# Autodesk Inventor assembly: Base-Rotation-Test
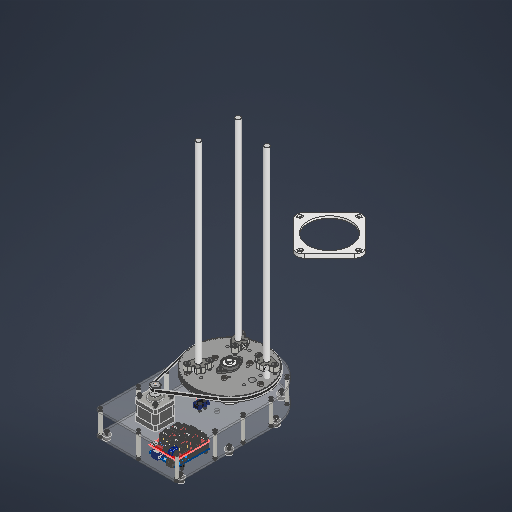
[picture p0: Inventor's stored thumbnail of the model, 512x512]
Saved by Autodesk Inventor 2025.2 (Build 292293000, 293)
## iProperties
Created: 2025-04-10
Part Number: Base-Rotation-Test
Document SubType Name: Assembly
Designer: Tiago
Author: Tiago
## Documents named in this file (32)
- C:\Users\Tiago\Documents\Inventor\Exp. Braço v1\Base-Rotation-Test.iam
- C:\Users\Tiago\Documents\Inventor\Exp. Braço v1\NEMA17 42-38.ipt
- C:\Users\Tiago\Documents\Inventor\Exp. Braço v1\Linear_Shaft_Support_SHF10.ipt
- C:\Users\Tiago\Documents\Inventor\Exp. Braço v1\rodshaft_10x400.ipt
- C:\Users\Tiago\Documents\Inventor\Exp. Braço v1\Arduino_CNC_Assembly.iam
- C:\Users\Tiago\Documents\Inventor\Exp. Braço v1\Base_solida_Down.ipt
- C:\Users\Tiago\Documents\Inventor\Exp. Braço v1\Amortecedor_Borracha.ipt
- C:\Users\Tiago\Documents\Inventor\Exp. Braço v1\Espaçador_m3_L3.5.ipt
- C:\Users\Tiago\Documents\Inventor\Exp. Braço v1\espaçador_M3_L40.ipt
- C:\Users\Tiago\Documents\Inventor\Exp. Braço v1\GT2Pulley_z20.ipt
- C:\Users\Tiago\Documents\Inventor\Exp. Braço v1\Base-Rotation\Design Accelerator\Synchronous Belts Transmission3.iam
- C:\Users\Tiago\Documents\Inventor\Exp. Braço v1\Anilha_M3.ipt
- C:\Users\Tiago\Documents\Inventor\Exp. Braço v1\M3 x0.5 ALT (...).ipt
- C:\Users\Tiago\Documents\Inventor\Exp. Braço v1\Porca_sextavada(4M).ipt
- C:\Users\Tiago\Documents\Inventor\Exp. Braço v1\M3 x8L_hexagonal_BigHEAD.ipt
- C:\Users\Tiago\Documents\Inventor\Exp. Braço v1\M3 x5L_hexagonal.ipt
- C:\Users\Tiago\Documents\Inventor\Exp. Braço v1\M4x22L_Hex.ipt
- C:\Users\Tiago\Documents\Inventor\Exp. Braço v1\M5 x12L_Hex_C.ipt
- M5 x12L_Hex_C.ipt
- C:\Users\Tiago\Documents\Inventor\Exp. Braço v1\M5x16L_Hex.ipt
- C:\Users\Tiago\Documents\Inventor\Exp. Braço v1\Porca_sextavada(3M).ipt
- C:\Users\Tiago\Documents\Inventor\Exp. Braço v1\M2x12L_Hex.ipt
- M2x12L_Hex.ipt
- C:\Users\Tiago\Documents\Inventor\Exp. Braço v1\Porca_sextavada(M2).ipt
- C:\Users\Tiago\Documents\Inventor\Exp. Braço v1\M5_nylonLock_Nut.ipt
- C:\Users\Tiago\Documents\Inventor\Exp. Braço v1\Limit switch\complete limit switch\complete limit switch\complete limit switch.ipt
- C:\Users\Tiago\Documents\Inventor\Exp. Braço v1\Base_solida_TestBR.ipt
- C:\Users\Tiago\Documents\Inventor\Exp. Braço v1\Rolamento TestBR\61814\61814\61814.iam
- C:\Users\Tiago\Documents\Inventor\Exp. Braço v1\Test_BR\Fix_bearing_Base.ipt
- C:\Users\Tiago\Documents\Inventor\Exp. Braço v1\PoliaDentada220dentes_TestBR.ipt
- C:\Users\Tiago\Documents\Inventor\Exp. Braço v1\Test_BR\Fix_toDown_bearing.ipt
- C:\Users\Tiago\Documents\Inventor\Exp. Braço v1\KFL08 - Mancal Flange oval Ø8_BRTest.ipt
## Components (124 placed, 29 different names)
1. NEMA17 42-38:1 — Mate:85, Mate:86, Flush:4, Mate:87, Flush:8
2. Linear_Shaft_Support_SHF10:1 — Mate:20, Insert:129, Insert:138, Insert:139
3. Linear_Shaft_Support_SHF10:2 — Mate:21, Mate:133, Insert:131, Insert:134, Insert:135
4. Linear_Shaft_Support_SHF10:3 — Mate:22, Insert:130, Insert:136, Insert:137
5. rodshaft_10x400:1 — Mate:22
6. rodshaft_10x400:2 — Mate:21, Mate:133
7. rodshaft_10x400:3 — Mate:20
8. Base_solida_TestBR:1 — Mate:31, Flush:1, Flush:2, Mate:85, Mate:87, Mate:97, Mate:98, Flush:8, Mate:107, Mate:111, Mate:112, Mate:113, Mate:117, Insert:150, Insert:151, Insert:162, Insert:163, Insert:164, Insert:165, Insert:166, Insert:167, Insert:168, Insert:169, Insert:170, Insert:171, Insert:172, Insert:173, Mate:184, Mate:185, Mate:186, Mate:190, Flush:9, Mate:192, Mate:193
9. Arduino_CNC_Assembly:1 [sub-assembly] — Mate:32, Mate:33, Mate:34, Mate:35, Mate:36, Insert:111, Insert:114, Insert:115, Insert:116
10. Base_solida_Down:1 — Mate:31, Flush:1, Flush:2, Mate:32, Mate:33, Mate:34, Mate:35, Mate:36, Mate:37, Mate:38, Mate:39, Mate:40, Mate:41, Mate:42, Mate:43, Mate:44, Mate:54, Mate:55, Mate:56, Mate:57, Mate:58, Mate:59, Mate:61, Mate:62, Mate:63, Mate:64, Mate:65, Mate:66, Mate:67, Mate:68, Mate:69, Mate:70, Mate:71, Mate:72, Mate:73, Mate:74, Mate:75, Mate:76, Mate:77, Mate:78, Mate:79, Mate:80, Mate:81, Mate:82, Mate:83, Mate:84, Flush:7, Mate:153, Mate:154, Insert:95, Insert:96, Mate:155, Mate:156, Mate:157, Mate:158, Mate:159, Mate:160, Mate:161, Mate:162, Insert:112, Insert:113, Insert:140, Insert:141, Insert:142, Insert:143, Insert:144, Insert:145, Insert:146, Insert:147, Insert:152, Insert:153, Insert:154, Insert:155, Insert:156, Insert:157, Insert:158, Insert:159, Insert:160, Insert:161, Insert:175, Insert:176
11. Amortecedor_Borracha:1 — Mate:57, Mate:159, Insert:102
12. Amortecedor_Borracha:2 — Mate:58, Mate:160, Insert:100
13. Amortecedor_Borracha:3 — Mate:59, Mate:161, Insert:99
14. Amortecedor_Borracha:4 — Mate:56, Mate:158, Insert:101
15. Amortecedor_Borracha:5 — Mate:153, Mate:162, Insert:98
16. Amortecedor_Borracha:6 — Mate:54, Mate:156, Mate:164
17. Amortecedor_Borracha:7 — Mate:154, Mate:155, Insert:97
18. Amortecedor_Borracha:8 — Mate:55, Mate:157, Mate:163
19. Espaçador_m3_L3.5:1 — Mate:37, Mate:41
20. Espaçador_m3_L3.5:2 — Mate:38, Mate:44
21. Espaçador_m3_L3.5:3 — Mate:40, Mate:42
22. Espaçador_m3_L3.5:4 — Mate:39, Mate:43
23. espaçador_M3_L40:1 — Mate:61, Mate:73
24. espaçador_M3_L40:2 — Mate:62, Mate:75
25. espaçador_M3_L40:3 — Mate:63, Mate:76
26. espaçador_M3_L40:4 — Mate:64, Mate:77
27. espaçador_M3_L40:5 — Mate:65, Mate:78
28. espaçador_M3_L40:6 — Mate:66, Mate:79
29. espaçador_M3_L40:7 — Mate:67, Mate:74
30. espaçador_M3_L40:8 — Mate:68, Mate:84
31. espaçador_M3_L40:9 — Mate:69, Mate:83
32. espaçador_M3_L40:10 — Mate:70, Mate:82
33. espaçador_M3_L40:11 — Mate:71, Mate:81
34. espaçador_M3_L40:12 — Mate:72, Mate:80
35. GT2Pulley_z20:1 — Mate:86, Flush:4, Mate:96, Flush:6
36. Synchronous Belts Transmission:1 [sub-assembly] — Mate:96, Flush:6
37. M3 x0.5 ALT (...):1 — Insert:162
38. M3 x0.5 ALT (...):2 — Insert:164
39. M3 x0.5 ALT (...):3 — Insert:165
40. M3 x0.5 ALT (...):4 — Insert:166
41. M3 x0.5 ALT (...):5 — Insert:167
42. M3 x0.5 ALT (...):6 — Insert:168
43. M3 x0.5 ALT (...):7 — Insert:169
44. M3 x0.5 ALT (...):8 — Insert:173
45. M3 x0.5 ALT (...):9 — Insert:172
46. M3 x0.5 ALT (...):10 — Insert:171
47. M3 x0.5 ALT (...):11 — Insert:170
48. M3 x0.5 ALT (...):12 — Insert:163
49. M3 x0.5 ALT (...):13 — Insert:156
50. M3 x0.5 ALT (...):14 — Insert:155
51. M3 x0.5 ALT (...):15 — Insert:154
52. M3 x0.5 ALT (...):16 — Insert:153
53. M3 x0.5 ALT (...):17 — Insert:152
54. M3 x0.5 ALT (...):18 — Insert:96
55. M3 x0.5 ALT (...):19 — Insert:161
56. M3 x0.5 ALT (...):20 — Insert:159
57. M3 x0.5 ALT (...):21 — Insert:160
58. M3 x0.5 ALT (...):22 — Insert:158
59. M3 x0.5 ALT (...):23 — Insert:157
60. M3 x0.5 ALT (...):24 — Insert:95
61. Anilha_M3:25 — Mate:107, Insert:106
62. Anilha_M3:26 — Mate:113, Insert:105
63. Anilha_M3:27 — Mate:112, Insert:104
64. Anilha_M3:28 — Mate:111, Insert:103
65. Porca_sextavada(4M):2 — Mate:117
66. KFL08 - Mancal Flange oval Ø8_BRTest:1 — Insert:133, Insert:174, Mate:202, Mate:203, Mate:204
67. M3 x0.5 ALT (...):29 — Insert:98
68. M3 x0.5 ALT (...):30 — Insert:97
69. M3 x0.5 ALT (...):31 — Insert:99
70. M3 x0.5 ALT (...):32 — Insert:100
71. M3 x0.5 ALT (...):33 — Insert:101
72. M3 x0.5 ALT (...):34 — Insert:102
73. M3 x0.5 ALT (...):35 — Mate:163
74. M3 x0.5 ALT (...):36 — Mate:164
75. M3 x8L_hexagonal_BigHEAD:1 — Insert:103
76. M3 x8L_hexagonal_BigHEAD:2 — Insert:104
77. M3 x8L_hexagonal_BigHEAD:3 — Insert:105
78. M3 x8L_hexagonal_BigHEAD:4 — Insert:106
79. M3 x5L_hexagonal:1 — Insert:175
80. M3 x5L_hexagonal:2 — Insert:176
81. M3 x5L_hexagonal:3 — Insert:112
82. M3 x5L_hexagonal:4 — Insert:113
83. M3 x5L_hexagonal:5 — Insert:111
84. M3 x5L_hexagonal:6 — Insert:114
85. M3 x5L_hexagonal:7 — Insert:115
86. M3 x5L_hexagonal:8 — Insert:116
87. M4x22L_Hex:1
88. M5 x12L_Hex_C:1 — Insert:129
89. M5 x12L_Hex_C:2 — Insert:130
90. M5 x12L_Hex_C:3 — Insert:131
91. M5x16L_Hex:1 — Insert:174
92. M5x16L_Hex:2 — Insert:133
93. M5x16L_Hex:3 — Insert:137
94. M5x16L_Hex:4 — Insert:135
95. M5x16L_Hex:5 — Insert:136
96. M5x16L_Hex:6 — Insert:139
97. M5x16L_Hex:7 — Insert:138
98. M5x16L_Hex:8 — Insert:134
99. Porca_sextavada(3M):1 — Insert:140
100. Porca_sextavada(3M):2 — Insert:142
101. Porca_sextavada(3M):3 — Insert:141
102. Porca_sextavada(3M):4 — Insert:143
103. Porca_sextavada(3M):5 — Insert:144
104. Porca_sextavada(3M):6 — Insert:147
105. Porca_sextavada(3M):7 — Insert:146
106. Porca_sextavada(3M):8 — Insert:145
107. M2x12L_Hex:1 — Insert:181
108. M2x12L_Hex:2 — Insert:182
109. Porca_sextavada(M2):1 — Insert:151
110. Porca_sextavada(M2):2 — Insert:150
111. M5_nylonLock_Nut:1
112. M5_nylonLock_Nut:2
113. M5_nylonLock_Nut:3
114. M5_nylonLock_Nut:4
115. M5_nylonLock_Nut:5
116. M5_nylonLock_Nut:6
117. M5_nylonLock_Nut:7
118. M5_nylonLock_Nut:8
119. PoliaDentada220dentes_TestBR:1 — Mate:197, Mate:199, Mate:201, Mate:202, Mate:203, Mate:204
120. complete limit switch:1 — Mate:184, Mate:185, Mate:186, Insert:181, Insert:182
121. 61814:1 [sub-assembly] — Mate:190, Flush:9, Mate:191, Mate:196, Mate:197, Mate:198, Mate:200
122. Fix_bearing_Base:1 — Mate:191, Mate:192, Mate:193, Mate:201
123. Fix_bearing_Base:2
124. Fix_toDown_bearing:1 — Mate:196, Mate:198, Mate:199, Mate:200
## Relationships (159: Mate 87, Insert 65, Flush 7)
- Mate:20: Linear_Shaft_Support_SHF10:1 ↔ rodshaft_10x400:3
- Mate:21: Linear_Shaft_Support_SHF10:2 ↔ rodshaft_10x400:2
- Mate:22: Linear_Shaft_Support_SHF10:3 ↔ rodshaft_10x400:1
- Mate:31 (40 mm): Base_solida_TestBR:1 ↔ Base_solida_Down:1
- Flush:1: Base_solida_TestBR:1 ↔ Base_solida_Down:1
- Flush:2: Base_solida_TestBR:1 ↔ Base_solida_Down:1
- Mate:32 (5 mm): Arduino_CNC_Assembly:1 ↔ Base_solida_Down:1
- Mate:33: Arduino_CNC_Assembly:1 ↔ Base_solida_Down:1
- Mate:34: Arduino_CNC_Assembly:1 ↔ Base_solida_Down:1
- Mate:35: Arduino_CNC_Assembly:1 ↔ Base_solida_Down:1
- Mate:36: Arduino_CNC_Assembly:1 ↔ Base_solida_Down:1
- Mate:37: Base_solida_Down:1 ↔ Espaçador_m3_L3.5:1
- Mate:38: Base_solida_Down:1 ↔ Espaçador_m3_L3.5:2
- Mate:39: Base_solida_Down:1 ↔ Espaçador_m3_L3.5:4
- Mate:40: Base_solida_Down:1 ↔ Espaçador_m3_L3.5:3
- Mate:41: Base_solida_Down:1 ↔ Espaçador_m3_L3.5:1
- Mate:42: Base_solida_Down:1 ↔ Espaçador_m3_L3.5:3
- Mate:43: Base_solida_Down:1 ↔ Espaçador_m3_L3.5:4
- Mate:44: Base_solida_Down:1 ↔ Espaçador_m3_L3.5:2
- Mate:54: Base_solida_Down:1 ↔ Amortecedor_Borracha:6
- Mate:55: Base_solida_Down:1 ↔ Amortecedor_Borracha:8
- Mate:56: Base_solida_Down:1 ↔ Amortecedor_Borracha:4
- Mate:57: Base_solida_Down:1 ↔ Amortecedor_Borracha:1
- Mate:58: Base_solida_Down:1 ↔ Amortecedor_Borracha:2
- Mate:59: Base_solida_Down:1 ↔ Amortecedor_Borracha:3
- Mate:61: Base_solida_Down:1 ↔ espaçador_M3_L40:1
- Mate:62: Base_solida_Down:1 ↔ espaçador_M3_L40:2
- Mate:63: Base_solida_Down:1 ↔ espaçador_M3_L40:3
- Mate:64: Base_solida_Down:1 ↔ espaçador_M3_L40:4
- Mate:65: Base_solida_Down:1 ↔ espaçador_M3_L40:5
- Mate:66: Base_solida_Down:1 ↔ espaçador_M3_L40:6
- Mate:67: Base_solida_Down:1 ↔ espaçador_M3_L40:7
- Mate:68: Base_solida_Down:1 ↔ espaçador_M3_L40:8
- Mate:69: Base_solida_Down:1 ↔ espaçador_M3_L40:9
- Mate:70: Base_solida_Down:1 ↔ espaçador_M3_L40:10
- Mate:71: Base_solida_Down:1 ↔ espaçador_M3_L40:11
- Mate:72: Base_solida_Down:1 ↔ espaçador_M3_L40:12
- Mate:73: Base_solida_Down:1 ↔ espaçador_M3_L40:1
- Mate:74: Base_solida_Down:1 ↔ espaçador_M3_L40:7
- Mate:75: Base_solida_Down:1 ↔ espaçador_M3_L40:2
- Mate:76: Base_solida_Down:1 ↔ espaçador_M3_L40:3
- Mate:77: Base_solida_Down:1 ↔ espaçador_M3_L40:4
- Mate:78: Base_solida_Down:1 ↔ espaçador_M3_L40:5
- Mate:79: Base_solida_Down:1 ↔ espaçador_M3_L40:6
- Mate:80: Base_solida_Down:1 ↔ espaçador_M3_L40:12
- Mate:81: Base_solida_Down:1 ↔ espaçador_M3_L40:11
- Mate:82: Base_solida_Down:1 ↔ espaçador_M3_L40:10
- Mate:83: Base_solida_Down:1 ↔ espaçador_M3_L40:9
- Mate:84: Base_solida_Down:1 ↔ espaçador_M3_L40:8
- Mate:85: NEMA17 42-38:1 ↔ Base_solida_TestBR:1
- Mate:86: NEMA17 42-38:1 ↔ GT2Pulley_z20:1
- Flush:4 (-0.8 mm): NEMA17 42-38:1 ↔ GT2Pulley_z20:1
- Mate:87: NEMA17 42-38:1 ↔ Base_solida_TestBR:1
- Mate:96: GT2Pulley_z20:1 ↔ Synchronous Belts Transmission:1
- Flush:6 (2 mm): GT2Pulley_z20:1 ↔ Synchronous Belts Transmission:1
- Flush:7: Base_solida_Down:1
- Mate:97: Base_solida_TestBR:1
- Mate:98: Base_solida_TestBR:1
- Flush:8 (59.286 mm): NEMA17 42-38:1 ↔ Base_solida_TestBR:1
- Mate:107: Base_solida_TestBR:1 ↔ Anilha_M3:25
- Mate:111: Base_solida_TestBR:1 ↔ Anilha_M3:28
- Mate:112: Base_solida_TestBR:1 ↔ Anilha_M3:27
- Mate:113: Base_solida_TestBR:1 ↔ Anilha_M3:26
- Mate:117: Base_solida_TestBR:1 ↔ Porca_sextavada(4M):2
- Mate:133: Linear_Shaft_Support_SHF10:2 ↔ rodshaft_10x400:2
- Mate:153: Base_solida_Down:1 ↔ Amortecedor_Borracha:5
- Mate:154: Base_solida_Down:1 ↔ Amortecedor_Borracha:7
- Insert:95: Base_solida_Down:1 ↔ M3 x0.5 ALT (...):24
- Insert:96: Base_solida_Down:1 ↔ M3 x0.5 ALT (...):18
- Mate:155: Base_solida_Down:1 ↔ Amortecedor_Borracha:7
- Insert:97: Amortecedor_Borracha:7 ↔ M3 x0.5 ALT (...):30
- Mate:156: Base_solida_Down:1 ↔ Amortecedor_Borracha:6
- Mate:157: Base_solida_Down:1 ↔ Amortecedor_Borracha:8
- Mate:158: Base_solida_Down:1 ↔ Amortecedor_Borracha:4
- Mate:159: Base_solida_Down:1 ↔ Amortecedor_Borracha:1
- Mate:160: Base_solida_Down:1 ↔ Amortecedor_Borracha:2
- Mate:161: Base_solida_Down:1 ↔ Amortecedor_Borracha:3
- Mate:162: Base_solida_Down:1 ↔ Amortecedor_Borracha:5
- Insert:98: Amortecedor_Borracha:5 ↔ M3 x0.5 ALT (...):29
- Insert:99: Amortecedor_Borracha:3 ↔ M3 x0.5 ALT (...):31
- Insert:100: Amortecedor_Borracha:2 ↔ M3 x0.5 ALT (...):32
- Insert:101: Amortecedor_Borracha:4 ↔ M3 x0.5 ALT (...):33
- Insert:102: Amortecedor_Borracha:1 ↔ M3 x0.5 ALT (...):34
- Mate:163: Amortecedor_Borracha:8 ↔ M3 x0.5 ALT (...):35
- Mate:164: Amortecedor_Borracha:6 ↔ M3 x0.5 ALT (...):36
- Insert:103: Anilha_M3:28 ↔ M3 x8L_hexagonal_BigHEAD:1
- Insert:104: Anilha_M3:27 ↔ M3 x8L_hexagonal_BigHEAD:2
- Insert:105: Anilha_M3:26 ↔ M3 x8L_hexagonal_BigHEAD:3
- Insert:106: Anilha_M3:25 ↔ M3 x8L_hexagonal_BigHEAD:4
- Insert:111: Arduino_CNC_Assembly:1 ↔ M3 x5L_hexagonal:5
- Insert:112: Base_solida_Down:1 ↔ M3 x5L_hexagonal:3
- Insert:113: Base_solida_Down:1 ↔ M3 x5L_hexagonal:4
- Insert:114: Arduino_CNC_Assembly:1 ↔ M3 x5L_hexagonal:6
- Insert:115: Arduino_CNC_Assembly:1 ↔ M3 x5L_hexagonal:7
- Insert:116: Arduino_CNC_Assembly:1 ↔ M3 x5L_hexagonal:8
- Insert:129: Linear_Shaft_Support_SHF10:1 ↔ M5 x12L_Hex_C:1
- Insert:130: Linear_Shaft_Support_SHF10:3 ↔ M5 x12L_Hex_C:2
- Insert:131: Linear_Shaft_Support_SHF10:2 ↔ M5 x12L_Hex_C:3
- Insert:133: KFL08 - Mancal Flange oval Ø8_BRTest:1 ↔ M5x16L_Hex:2
- Insert:134: Linear_Shaft_Support_SHF10:2 ↔ M5x16L_Hex:8
- Insert:135: Linear_Shaft_Support_SHF10:2 ↔ M5x16L_Hex:4
- Insert:136: Linear_Shaft_Support_SHF10:3 ↔ M5x16L_Hex:5
- Insert:137: Linear_Shaft_Support_SHF10:3 ↔ M5x16L_Hex:3
- Insert:138: Linear_Shaft_Support_SHF10:1 ↔ M5x16L_Hex:7
- Insert:139: Linear_Shaft_Support_SHF10:1 ↔ M5x16L_Hex:6
- Insert:140: Base_solida_Down:1 ↔ Porca_sextavada(3M):1
- Insert:141: Base_solida_Down:1 ↔ Porca_sextavada(3M):3
- Insert:142: Base_solida_Down:1 ↔ Porca_sextavada(3M):2
- Insert:143: Base_solida_Down:1 ↔ Porca_sextavada(3M):4
- Insert:144: Base_solida_Down:1 ↔ Porca_sextavada(3M):5
- Insert:145: Base_solida_Down:1 ↔ Porca_sextavada(3M):8
- Insert:146: Base_solida_Down:1 ↔ Porca_sextavada(3M):7
- Insert:147: Base_solida_Down:1 ↔ Porca_sextavada(3M):6
- Insert:150: Base_solida_TestBR:1 ↔ Porca_sextavada(M2):2
- Insert:151: Base_solida_TestBR:1 ↔ Porca_sextavada(M2):1
- Insert:152: Base_solida_Down:1 ↔ M3 x0.5 ALT (...):17
- Insert:153: Base_solida_Down:1 ↔ M3 x0.5 ALT (...):16
- Insert:154: Base_solida_Down:1 ↔ M3 x0.5 ALT (...):15
- Insert:155: Base_solida_Down:1 ↔ M3 x0.5 ALT (...):14
- Insert:156: Base_solida_Down:1 ↔ M3 x0.5 ALT (...):13
- Insert:157: Base_solida_Down:1 ↔ M3 x0.5 ALT (...):23
- Insert:158: Base_solida_Down:1 ↔ M3 x0.5 ALT (...):22
- Insert:159: Base_solida_Down:1 ↔ M3 x0.5 ALT (...):20
- Insert:160: Base_solida_Down:1 ↔ M3 x0.5 ALT (...):21
- Insert:161: Base_solida_Down:1 ↔ M3 x0.5 ALT (...):19
- Insert:162: Base_solida_TestBR:1 ↔ M3 x0.5 ALT (...):1
- Insert:163: Base_solida_TestBR:1 ↔ M3 x0.5 ALT (...):12
- Insert:164: Base_solida_TestBR:1 ↔ M3 x0.5 ALT (...):2
- Insert:165: Base_solida_TestBR:1 ↔ M3 x0.5 ALT (...):3
- Insert:166: Base_solida_TestBR:1 ↔ M3 x0.5 ALT (...):4
- Insert:167: Base_solida_TestBR:1 ↔ M3 x0.5 ALT (...):5
- Insert:168: Base_solida_TestBR:1 ↔ M3 x0.5 ALT (...):6
- Insert:169: Base_solida_TestBR:1 ↔ M3 x0.5 ALT (...):7
- Insert:170: Base_solida_TestBR:1 ↔ M3 x0.5 ALT (...):11
- Insert:171: Base_solida_TestBR:1 ↔ M3 x0.5 ALT (...):10
- Insert:172: Base_solida_TestBR:1 ↔ M3 x0.5 ALT (...):9
- Insert:173: Base_solida_TestBR:1 ↔ M3 x0.5 ALT (...):8
- Insert:174: KFL08 - Mancal Flange oval Ø8_BRTest:1 ↔ M5x16L_Hex:1
- Insert:175: Base_solida_Down:1 ↔ M3 x5L_hexagonal:1
- Insert:176: Base_solida_Down:1 ↔ M3 x5L_hexagonal:2
- Mate:184: Base_solida_TestBR:1 ↔ complete limit switch:1
- Mate:185: Base_solida_TestBR:1 ↔ complete limit switch:1
- Mate:186: Base_solida_TestBR:1 ↔ complete limit switch:1
- Insert:181: M2x12L_Hex:1 ↔ complete limit switch:1
- Insert:182: M2x12L_Hex:2 ↔ complete limit switch:1
- Mate:190: Base_solida_TestBR:1 ↔ 61814:1
- Flush:9 (-3 mm): Base_solida_TestBR:1 ↔ 61814:1
- Mate:191: 61814:1 ↔ Fix_bearing_Base:1
- Mate:192: Base_solida_TestBR:1 ↔ Fix_bearing_Base:1
- Mate:193: Base_solida_TestBR:1 ↔ Fix_bearing_Base:1
- Mate:196: 61814:1 ↔ Fix_toDown_bearing:1
- Mate:197: PoliaDentada220dentes_TestBR:1 ↔ 61814:1
- Mate:198: 61814:1 ↔ Fix_toDown_bearing:1
- Mate:199: PoliaDentada220dentes_TestBR:1 ↔ Fix_toDown_bearing:1
- Mate:200: 61814:1 ↔ Fix_toDown_bearing:1
- Mate:201: PoliaDentada220dentes_TestBR:1 ↔ Fix_bearing_Base:1
- Mate:202: KFL08 - Mancal Flange oval Ø8_BRTest:1 ↔ PoliaDentada220dentes_TestBR:1
- Mate:203: KFL08 - Mancal Flange oval Ø8_BRTest:1 ↔ PoliaDentada220dentes_TestBR:1
- Mate:204: KFL08 - Mancal Flange oval Ø8_BRTest:1 ↔ PoliaDentada220dentes_TestBR:1
